# Autodesk Inventor assembly: Herramienta 1
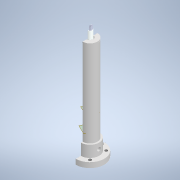
[picture p0: Inventor's stored thumbnail of the model, 180x180]
Saved by Autodesk Inventor 2022 (Build 260153000, 153)
## iProperties
Created: 2022-08-26
Part Number: Herramienta 1
Document SubType Name: Assembly
Designer: David
Author: David
## Documents named in this file (8)
- C:\Users\David\OneDrive\Documentos\Universidad\Decimo Semestre\Robotica\Lab 1\Herramienta 1.iam
- C:\Users\David\OneDrive\Documentos\Universidad\Decimo Semestre\Robotica\Lab 1\Brida para herramienta - Copy.ipt
- C:\Users\David\OneDrive\Documentos\Universidad\Decimo Semestre\Robotica\Lab 1\Coil.ipt
- C:\Users\David\OneDrive\Documentos\Universidad\Decimo Semestre\Robotica\Lab 1\Soporte de Marcador.ipt
- C:\Users\David\OneDrive\Documentos\Universidad\Decimo Semestre\Robotica\Lab 1\expo-marker-1.snapshot.2\EM-COMPLETED MARKER.iam
- C:\Users\David\OneDrive\Documentos\Universidad\Decimo Semestre\Robotica\Lab 1\Acople Resorte-Marcador.ipt
- C:\Users\David\OneDrive\Documentos\Universidad\Decimo Semestre\Robotica\Lab 1\Tapa.ipt
- C:\Users\David\OneDrive\Documentos\Universidad\Decimo Semestre\Robotica\Lab 1\Soporte Resorte.ipt
## Components (7 placed, 7 different names)
1. Brida para herramienta - Copy:1 — Mate:2, Mate:3, Mate:17
2. Coil:1 — Mate:4, Flush:1, Mate:8
3. Soporte de Marcador:1 — Mate:1, Mate:2, Mate:3, Mate:4, Mate:5, Mate:7, Mate:9, Mate:11, Mate:13, Mate:14, Mate:15, Mate:16, Mate:17
4. EM-COMPLETED MARKER:1 [sub-assembly] — Mate:1, Mate:6
5. Acople Resorte-Marcador:1 — Mate:5, Mate:6, Flush:1, Mate:14
6. Soporte Resorte:6 — Mate:7, Mate:8, Mate:13, Mate:15
7. Tapa:1 — Mate:9, Mate:11, Mate:16
## Relationships (16: Mate 15, Flush 1)
- Mate:1: Soporte de Marcador:1 ↔ EM-COMPLETED MARKER:1
- Mate:2: Brida para herramienta - Copy:1 ↔ Soporte de Marcador:1
- Mate:3: Brida para herramienta - Copy:1 ↔ Soporte de Marcador:1
- Mate:4: Coil:1 ↔ Soporte de Marcador:1
- Mate:5: Soporte de Marcador:1 ↔ Acople Resorte-Marcador:1
- Mate:6: EM-COMPLETED MARKER:1 ↔ Acople Resorte-Marcador:1
- Flush:1: Coil:1 ↔ Acople Resorte-Marcador:1
- Mate:7: Soporte de Marcador:1 ↔ Soporte Resorte:6
- Mate:8: Coil:1 ↔ Soporte Resorte:6
- Mate:9: Soporte de Marcador:1 ↔ Tapa:1
- Mate:11: Soporte de Marcador:1 ↔ Tapa:1
- Mate:13: Soporte de Marcador:1 ↔ Soporte Resorte:6
- Mate:14 (0.75 mm): Soporte de Marcador:1 ↔ Acople Resorte-Marcador:1
- Mate:15 (0.75 mm): Soporte de Marcador:1 ↔ Soporte Resorte:6
- Mate:16 (0.75 mm): Soporte de Marcador:1 ↔ Tapa:1
- Mate:17: Brida para herramienta - Copy:1 ↔ Soporte de Marcador:1
